# Autodesk Inventor assembly: Assembly1
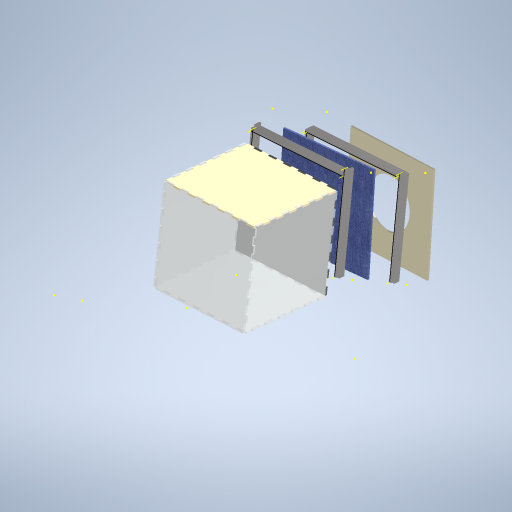
[picture p0: Inventor's stored thumbnail of the model, 512x512]
Saved by Autodesk Inventor 2024 (Build 280153000, 153)
## iProperties
Created: 2023-10-19
Part Number: Assembly1
Document SubType Name: Assembly
Designer: liuyu
Author: liuyu
## Documents named in this file (5)
- C:\Users\liuyu\Desktop\NUS\Y4S1\IoT182FYP\Prototype\3D Design\Assembly1.iam
- C:\Users\liuyu\Desktop\NUS\Y4S1\IoT182FYP\Prototype\3D Design\Part1.ipt
- C:\Users\liuyu\Desktop\NUS\Y4S1\IoT182FYP\Prototype\3D Design\Part2.ipt
- C:\Users\liuyu\Desktop\NUS\Y4S1\IoT182FYP\Prototype\3D Design\Part3.ipt
- C:\Users\liuyu\Desktop\NUS\Y4S1\IoT182FYP\Prototype\3D Design\Part5.ipt
## Components (14 placed, 4 different names)
1. Part1:1 — Mate:1, Mate:2, Mate:3, Mate:4, Mate:5, Mate:7, Mate:8
2. Part1:2 — Mate:1, Mate:2, Mate:6
3. Part1:3 — Mate:3, Mate:4, Mate:5, Mate:6, Mate:11, Mate:12, Mate:13
4. Part1:4 — Mate:9, Mate:10, Mate:18, Mate:21
5. Part1:5 — Mate:7, Mate:8, Mate:9, Mate:10
6. Part1:6 — Mate:11, Mate:12, Mate:14, Mate:22
7. Part2:2 — Mate:17, Mate:18, Mate:19, Mate:20, Mate:21, Mate:22
8. Part2:4 — Mate:15, Mate:16
9. Part2:5 — Mate:13, Mate:14, Mate:15, Mate:16, Mate:17, Mate:19, Mate:20
10. Part2:6
11. Part2:7
12. Part2:8
13. Part3:1
14. Part5:1
## Relationships (27: Mate 27)
- Mate:1: Part1:1 ↔ Part1:2
- Mate:2: Part1:1 ↔ Part1:2
- Mate:3: Part1:1 ↔ Part1:3
- Mate:4: Part1:1 ↔ Part1:3
- Mate:5: Part1:1 ↔ Part1:3
- Mate:6: Part1:2 ↔ Part1:3
- Mate:7: Part1:1 ↔ Part1:5
- Mate:8: Part1:1 ↔ Part1:5
- Mate:9: Part1:4 ↔ Part1:5
- Mate:10: Part1:4 ↔ Part1:5
- Mate:11: Part1:3 ↔ Part1:6
- Mate:12: Part1:3 ↔ Part1:6
- Mate:13: Part1:3 ↔ Part2:5
- Mate:14: Part1:6 ↔ Part2:5
- Mate:15: Part2:4 ↔ Part2:5
- Mate:16: Part2:4 ↔ Part2:5
- Mate:17: Part2:2 ↔ Part2:5
- Mate:18: Part1:4 ↔ Part2:2
- Mate:19: Part2:2 ↔ Part2:5
- Mate:20: Part2:2 ↔ Part2:5
- Mate:21: Part1:4 ↔ Part2:2
- Mate:22: Part1:6 ↔ Part2:2
- [Mate]: Part2:7 ↔ Part2:8
- [Mate]: Part2:7 ↔ Part2:8
- [Mate]: Part2:6 ↔ Part2:8
- [Mate]: Part2:6 ↔ Part2:8
- [Mate]: Part2:6 ↔ Part2:8
## Named parameters: d34_d19 = 0 mm, d35_d20 = 0 mm, d36_d21 = 0 mm, d37_d23 = 0 mm, d38_d24 = 0 mm
